# Autodesk Inventor assembly: Finger
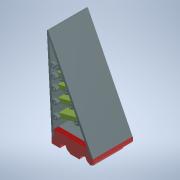
[picture p0: Inventor's stored thumbnail of the model, 180x180]
Saved by Autodesk Inventor 2021 (Build 250183000, 183)
## iProperties
Created: 2020-03-10
Part Number: Finger
Document SubType Name: Assembly
Designer: JochenAlt
Author: JochenAlt
## Documents named in this file (3)
- C:\Users\Jochen Alt\Documents\Daten\Projects\MiniBot\CAD\gripper\Finger.iam
- C:\Users\Jochen Alt\Documents\Daten\Projects\MiniBot\CAD\gripper\FingerEnclosure.ipt
- C:\Users\Jochen Alt\Documents\Daten\Projects\MiniBot\CAD\gripper\FinrayShaft.ipt
## Components (11 placed, 2 different names)
1. FingerEnclosure:1 — Mate:1, Mate:2, Mate:3, Mate:4, Mate:5, Mate:6, Mate:7, Mate:8, Mate:9, Mate:10, Mate:11, Mate:12, Mate:13, Mate:14, Mate:15, Mate:16, Mate:17, Mate:18, Mate:19, Mate:20
2. FinrayShaft:1 — Mate:6, Mate:15
3. FinrayShaft:2 — Mate:8, Mate:17
4. FinrayShaft:3 — Mate:9, Mate:20
5. FinrayShaft:4 — Mate:10, Mate:19
6. FinrayShaft:6 — Mate:7, Mate:18
7. FinrayShaft:7 — Mate:2, Mate:13
8. FinrayShaft:8 — Mate:3, Mate:14
9. FinrayShaft:9 — Mate:5, Mate:16
10. FinrayShaft:10 — Mate:4, Mate:11
11. FinrayShaft:11 — Mate:1, Mate:12
## Relationships (20: Mate 20)
- Mate:1: FingerEnclosure:1 ↔ FinrayShaft:11
- Mate:2: FingerEnclosure:1 ↔ FinrayShaft:7
- Mate:3: FingerEnclosure:1 ↔ FinrayShaft:8
- Mate:4: FingerEnclosure:1 ↔ FinrayShaft:10
- Mate:5: FingerEnclosure:1 ↔ FinrayShaft:9
- Mate:6: FingerEnclosure:1 ↔ FinrayShaft:1
- Mate:7: FingerEnclosure:1 ↔ FinrayShaft:6
- Mate:8: FingerEnclosure:1 ↔ FinrayShaft:2
- Mate:9: FingerEnclosure:1 ↔ FinrayShaft:3
- Mate:10: FingerEnclosure:1 ↔ FinrayShaft:4
- Mate:11: FingerEnclosure:1 ↔ FinrayShaft:10
- Mate:12: FingerEnclosure:1 ↔ FinrayShaft:11
- Mate:13: FingerEnclosure:1 ↔ FinrayShaft:7
- Mate:14: FingerEnclosure:1 ↔ FinrayShaft:8
- Mate:15: FingerEnclosure:1 ↔ FinrayShaft:1
- Mate:16: FingerEnclosure:1 ↔ FinrayShaft:9
- Mate:17: FingerEnclosure:1 ↔ FinrayShaft:2
- Mate:18: FingerEnclosure:1 ↔ FinrayShaft:6
- Mate:19: FingerEnclosure:1 ↔ FinrayShaft:4
- Mate:20: FingerEnclosure:1 ↔ FinrayShaft:3
